# Autodesk Inventor assembly: nhk41
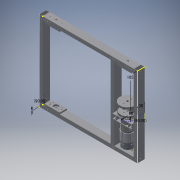
[picture p0: Inventor's stored thumbnail of the model, 180x180]
Saved by Autodesk Inventor 2019 (Build 230136000, 136)
## iProperties
Created: 2022-02-27
Part Number: nhk41
Material: 一般
Document SubType Name: Assembly
Designer: yuta
Author: yuta
## Documents named in this file (7)
- C:\Users\yuta\Documents\NHK\nhk41.iam
- C:\Users\yuta\Documents\NHK\nhk37.iam
- C:\Users\yuta\Documents\NHK\nhk40.ipt
- C:\Users\yuta\Documents\NHK\nhk43.ipt
- C:\Users\yuta\Documents\NHK\nhk39.ipt
- C:\Users\yuta\Documents\NHK\nhk48.ipt
- C:\Users\yuta\Documents\NHK\nhk45.ipt
## Components (9 placed, 6 different names)
1. nhk37:1 [sub-assembly] — メイト:1, メイト:2, メイト:3, メイト:8
2. nhk40:1 — メイト:1, メイト:2, メイト:3, メイト:4, フラッシュ:1, フラッシュ:2, メイト:5, フラッシュ:3, フラッシュ:4
3. nhk43:1 — メイト:4, フラッシュ:1, フラッシュ:2, メイト:6, フラッシュ:5, フラッシュ:6, メイト:9, フラッシュ:8, メイト:13, メイト:14, フラッシュ:9
4. nhk43:2 — メイト:5, フラッシュ:3, フラッシュ:4, メイト:7, フラッシュ:7, メイト:11, メイト:12
5. nhk39:1 — メイト:6, フラッシュ:5, フラッシュ:6
6. nhk48:1 — メイト:7, フラッシュ:7, メイト:8, メイト:10
7. nhk45:1 — メイト:9, フラッシュ:8, メイト:10
8. nhk45:2 — メイト:11, メイト:12
9. nhk45:3 — メイト:13, メイト:14, フラッシュ:9
## Relationships (23: Mate 14, Flush 9)
- メイト:1 [Mate]: nhk37:1 ↔ nhk40:1
- メイト:2 [Mate]: nhk37:1 ↔ nhk40:1
- メイト:3 [Mate]: nhk37:1 ↔ nhk40:1
- メイト:4 [Mate]: nhk40:1 ↔ nhk43:1
- フラッシュ:1 [Flush]: nhk40:1 ↔ nhk43:1
- フラッシュ:2 [Flush]: nhk40:1 ↔ nhk43:1
- メイト:5 [Mate]: nhk40:1 ↔ nhk43:2
- フラッシュ:3 [Flush]: nhk40:1 ↔ nhk43:2
- フラッシュ:4 [Flush]: nhk40:1 ↔ nhk43:2
- メイト:6 [Mate]: nhk43:1 ↔ nhk39:1
- フラッシュ:5 [Flush]: nhk43:1 ↔ nhk39:1
- フラッシュ:6 [Flush]: nhk43:1 ↔ nhk39:1
- メイト:7 [Mate]: nhk43:2 ↔ nhk48:1
- フラッシュ:7 [Flush]: nhk43:2 ↔ nhk48:1
- メイト:8 [Mate]: nhk37:1 ↔ nhk48:1
- メイト:9 [Mate]: nhk43:1 ↔ nhk45:1
- フラッシュ:8 [Flush]: nhk43:1 ↔ nhk45:1
- メイト:10 [Mate] (10 mm): nhk48:1 ↔ nhk45:1
- メイト:11 [Mate]: nhk43:2 ↔ nhk45:2
- メイト:12 [Mate]: nhk43:2 ↔ nhk45:2
- メイト:13 [Mate]: nhk43:1 ↔ nhk45:3
- メイト:14 [Mate]: nhk43:1 ↔ nhk45:3
- フラッシュ:9 [Flush]: nhk43:1 ↔ nhk45:3
